# Autodesk Inventor assembly: MTi-600 DEV assembly
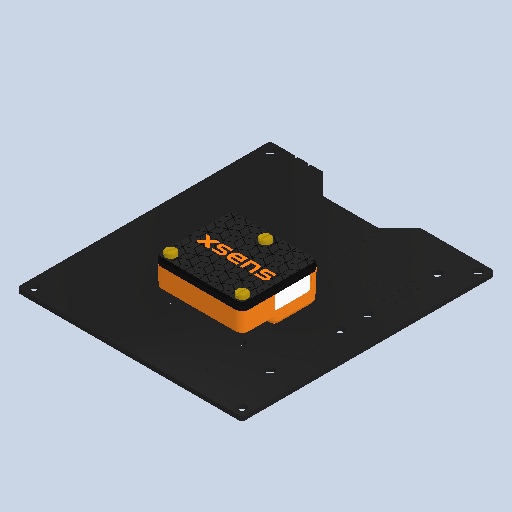
[picture p0: Inventor's stored thumbnail of the model, 512x512]
Saved by Autodesk Inventor 2023 (Build 270158000, 158)
## iProperties
Created: 2019-12-18
Part Number: MTi-600 DEV assembly
Description: STEP AP214
Document SubType Name: Assembly
Designer: ps737
Sending System: SolidWorks 2019
Preprocessor: SwSTEP 2.0
Title: MTi-600 DEV assembly.STEP
Revision Number: ANY
## Documents named in this file (4)
- C:\Users\ps737\OneDrive\바탕 화면\2024 ERP42\MTi 600-series STEP files\MTi-600 DEV assembly.iam
- C:\Users\ps737\OneDrive\바탕 화면\2024 ERP42\MTi 600-series STEP files\MTi-600 Assembly.iam
- C:\Users\ps737\OneDrive\바탕 화면\2024 ERP42\MTi 600-series STEP files\ISO 1580 - M2 x 10 --- 10N_ISO 1580 - M2 x 10 --- 10N.ipt
- C:\Users\ps737\OneDrive\바탕 화면\2024 ERP42\MTi 600-series STEP files\MTi-600 DEV Open CASCADE STEP translator 6.8 2.1.1.1.ipt
## Components (5 placed, 3 different names)
1. MTi-600 DEV Open CASCADE STEP translator 6.8 2.1.1.1:1 — 플러쉬:1, 메이트:8, 메이트:9, 메이트:10, 메이트:11
2. MTi-600 Assembly:2 [sub-assembly] — 메이트:1, 메이트:2, 메이트:3, 메이트:4, 메이트:5, 메이트:6, 플러쉬:1
3. ISO 1580 - M2 x 10 --- 10N_ISO 1580 - M2 x 10 --- 10N:4 — 메이트:3, 메이트:5, 메이트:8, 메이트:9
4. ISO 1580 - M2 x 10 --- 10N_ISO 1580 - M2 x 10 --- 10N:5 — 메이트:2, 메이트:6, 메이트:10, 메이트:11
5. ISO 1580 - M2 x 10 --- 10N_ISO 1580 - M2 x 10 --- 10N:6 — 메이트:1, 메이트:4
## Relationships (11: Mate 10, Flush 1)
- 메이트:1 [Mate]: MTi-600 Assembly:2 ↔ ISO 1580 - M2 x 10 --- 10N_ISO 1580 - M2 x 10 --- 10N:6
- 메이트:2 [Mate]: MTi-600 Assembly:2 ↔ ISO 1580 - M2 x 10 --- 10N_ISO 1580 - M2 x 10 --- 10N:5
- 메이트:3 [Mate]: MTi-600 Assembly:2 ↔ ISO 1580 - M2 x 10 --- 10N_ISO 1580 - M2 x 10 --- 10N:4
- 메이트:4 [Mate]: MTi-600 Assembly:2 ↔ ISO 1580 - M2 x 10 --- 10N_ISO 1580 - M2 x 10 --- 10N:6
- 메이트:5 [Mate]: MTi-600 Assembly:2 ↔ ISO 1580 - M2 x 10 --- 10N_ISO 1580 - M2 x 10 --- 10N:4
- 메이트:6 [Mate]: MTi-600 Assembly:2 ↔ ISO 1580 - M2 x 10 --- 10N_ISO 1580 - M2 x 10 --- 10N:5
- 플러쉬:1 [Flush] (-14.5 mm): MTi-600 DEV Open CASCADE STEP translator 6.8 2.1.1.1:1 ↔ MTi-600 Assembly:2
- 메이트:8 [Mate]: MTi-600 DEV Open CASCADE STEP translator 6.8 2.1.1.1:1 ↔ ISO 1580 - M2 x 10 --- 10N_ISO 1580 - M2 x 10 --- 10N:4
- 메이트:9 [Mate]: MTi-600 DEV Open CASCADE STEP translator 6.8 2.1.1.1:1 ↔ ISO 1580 - M2 x 10 --- 10N_ISO 1580 - M2 x 10 --- 10N:4
- 메이트:10 [Mate]: MTi-600 DEV Open CASCADE STEP translator 6.8 2.1.1.1:1 ↔ ISO 1580 - M2 x 10 --- 10N_ISO 1580 - M2 x 10 --- 10N:5
- 메이트:11 [Mate]: MTi-600 DEV Open CASCADE STEP translator 6.8 2.1.1.1:1 ↔ ISO 1580 - M2 x 10 --- 10N_ISO 1580 - M2 x 10 --- 10N:5
